# Autodesk Inventor assembly: top_ass_1
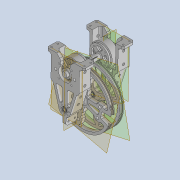
[picture p0: Inventor's stored thumbnail of the model, 180x180]
Saved by Autodesk Inventor 2020 (Build 240168000, 168)
## iProperties
Created: 2021-10-25
Part Number: top_ass_1
Document SubType Name: Assembly
Designer: Shuang Peng
Author: Shuang Peng
## Documents named in this file (2)
- D:\projects-3\torque fb tip\hardware\hapkit_1\top_ass_1.iam
- D:\projects-3\torque fb tip\hardware\hapkit_1\reducer_unit.iam
## Components (2 placed, 1 different names)
1. reducer_unit:1 [sub-assembly] — Flush:1, Mate:1, Flush:2
2. reducer_unit:2 [sub-assembly] — Flush:1, Mate:1, Flush:2
## Relationships (3: Flush 2, Mate 1)
- Flush:1: reducer_unit:1 ↔ reducer_unit:2
- Mate:1 (7 mm): reducer_unit:1 ↔ reducer_unit:2
- Flush:2: reducer_unit:1 ↔ reducer_unit:2
